# Autodesk Inventor assembly: eye_tracker_angled_assembly
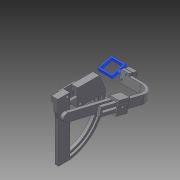
[picture p0: Inventor's stored thumbnail of the model, 180x180]
Saved by Autodesk Inventor 2015 (Build 190159000, 159)
## iProperties
Created: 2015-06-20
Part Number: eye_tracker_angled_assembly
Document SubType Name: Assembly
Designer: Master
Author: Master
## Documents named in this file (10)
- C:\Users\Master\Desktop\Alex_eye_tracker\eye_tracker_angled_assembly.iam
- C:\Users\Master\Desktop\Alex_eye_tracker\eye_cam_angled_bracket.ipt
- C:\Users\Master\Desktop\Alex_eye_tracker\eye_tracker_angled_arm.ipt
- C:\Users\Master\Desktop\Alex_eye_tracker\angled_arm_brace.ipt
- C:\Users\Master\Desktop\Alex_eye_tracker\eye_cam_arm_brace.ipt
- C:\Users\Master\Desktop\Alex_eye_tracker\eye_cam_arm.ipt
- C:\Users\Master\Desktop\Alex_eye_tracker\eye_cam_clamp.ipt
- C:\Users\Master\Desktop\Alex_eye_tracker\eye_cam_holder.ipt
- C:\Users\Master\Desktop\Alex_eye_tracker\top_plate.ipt
- C:\Users\Master\Desktop\Alex_eye_tracker\arm_plate.ipt
## Components (9 placed, 9 different names)
1. eye_cam_angled_bracket:1 — Mate:1, Insert:1, Mate:2, Tangent:1, Flush:7
2. eye_tracker_angled_arm:1 — Mate:1, Insert:1, Flush:1, Mate:3, Flush:2, Mate:6, Flush:4
3. angled_arm_brace:1 — Mate:2, Flush:1, Tangent:1
4. eye_cam_arm_brace:1 — Mate:3, Flush:2, Mate:5, Mate:6, Flush:3, Flush:8, Mate:10
5. eye_cam_arm:1 — Mate:5, Flush:3, Flush:4, Flush:5, Flush:6, Mate:7, Mate:9
6. eye_cam_clamp:1 — Flush:5, Flush:6, Mate:7, Mate:8
7. eye_cam_holder:1 — Mate:8
8. top_plate:1 — Flush:7
9. arm_plate:1 — Mate:9, Flush:8, Mate:10
## Relationships (19: Mate 9, Flush 8, Insert 1, Tangent 1)
- Mate:1: eye_cam_angled_bracket:1 ↔ eye_tracker_angled_arm:1
- Insert:1: eye_cam_angled_bracket:1 ↔ eye_tracker_angled_arm:1
- Mate:2: eye_cam_angled_bracket:1 ↔ angled_arm_brace:1
- Flush:1: eye_tracker_angled_arm:1 ↔ angled_arm_brace:1
- Tangent:1: eye_cam_angled_bracket:1 ↔ angled_arm_brace:1
- Mate:3: eye_tracker_angled_arm:1 ↔ eye_cam_arm_brace:1
- Flush:2: eye_tracker_angled_arm:1 ↔ eye_cam_arm_brace:1
- Mate:5: eye_cam_arm_brace:1 ↔ eye_cam_arm:1
- Mate:6: eye_tracker_angled_arm:1 ↔ eye_cam_arm_brace:1
- Flush:3 (-20 mm): eye_cam_arm_brace:1 ↔ eye_cam_arm:1
- Flush:4: eye_tracker_angled_arm:1 ↔ eye_cam_arm:1
- Flush:5: eye_cam_arm:1 ↔ eye_cam_clamp:1
- Flush:6: eye_cam_arm:1 ↔ eye_cam_clamp:1
- Mate:7 (0.5 mm): eye_cam_arm:1 ↔ eye_cam_clamp:1
- Mate:8: eye_cam_clamp:1 ↔ eye_cam_holder:1
- Flush:7: eye_cam_angled_bracket:1 ↔ top_plate:1
- Mate:9: eye_cam_arm:1 ↔ arm_plate:1
- Flush:8: eye_cam_arm_brace:1 ↔ arm_plate:1
- Mate:10 (0.25 mm): eye_cam_arm_brace:1 ↔ arm_plate:1
